# Autodesk Inventor assembly: Assemblyall
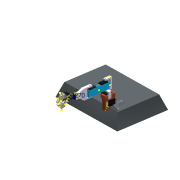
[picture p0: Inventor's stored thumbnail of the model, 180x180]
Saved by Autodesk Inventor 2022 (Build 260153000, 153)
## iProperties
Created: 2021-06-23
Part Number: Assemblyall
Document SubType Name: Assembly
Designer: athar
Author: athar
## Documents named in this file (16)
- C:\Users\Prajwal Patil\Desktop\HumanArmMimicBot-main\HumanArmMimicBot-main\AssemblyAlpha\Assemblyall.iam
- C:\Users\Prajwal Patil\Desktop\HumanArmMimicBot-main\HumanArmMimicBot-main\AssemblyAlpha\Part1_New.ipt
- C:\Users\Prajwal Patil\Desktop\HumanArmMimicBot-main\HumanArmMimicBot-main\AssemblyAlpha\Hand1.ipt
- C:\Users\Prajwal Patil\Desktop\HumanArmMimicBot-main\HumanArmMimicBot-main\AssemblyAlpha\Hand4.ipt
- C:\Users\Prajwal Patil\Desktop\HumanArmMimicBot-main\HumanArmMimicBot-main\AssemblyAlpha\Non Colour Claw.ipt
- C:\Users\Prajwal Patil\Desktop\HumanArmMimicBot-main\HumanArmMimicBot-main\AssemblyAlpha\Part1.ipt
- C:\Users\Prajwal Patil\Desktop\HumanArmMimicBot-main\HumanArmMimicBot-main\AssemblyAlpha\Part2.ipt
- C:\Users\Prajwal Patil\Desktop\HumanArmMimicBot-main\HumanArmMimicBot-main\AssemblyAlpha\Part4.ipt
- C:\Users\Prajwal Patil\Desktop\HumanArmMimicBot-main\HumanArmMimicBot-main\AssemblyAlpha\Part5.ipt
- C:\Users\Prajwal Patil\Desktop\HumanArmMimicBot-main\HumanArmMimicBot-main\AssemblyAlpha\motorshaft.ipt
- C:\Users\Prajwal Patil\Desktop\HumanArmMimicBot-main\HumanArmMimicBot-main\AssemblyAlpha\CSN EN ISO 8733 - 8x18-St.ipt
- C:\Users\Prajwal Patil\Desktop\HumanArmMimicBot-main\HumanArmMimicBot-main\AssemblyAlpha\Spur Gears2.iam
- C:\Users\Prajwal Patil\Desktop\HumanArmMimicBot-main\HumanArmMimicBot-main\AssemblyAlpha\bigServo_Derived.ipt
- C:\Users\Prajwal Patil\Desktop\HumanArmMimicBot-main\HumanArmMimicBot-main\AssemblyAlpha\Small_ServoDerived.ipt
- C:\Users\Prajwal Patil\Desktop\HumanArmMimicBot-main\HumanArmMimicBot-main\AssemblyAlpha\JIS B 1111 - M4x50.ipt
- C:\Users\Prajwal Patil\Desktop\HumanArmMimicBot-main\HumanArmMimicBot-main\AssemblyAlpha\base.ipt
## Components (68 placed, 15 different names)
1. Hand1:1 — Rotational:1, Rotational:2, Rotational:28, Mate:9, Rigid:18, Rotational:54
2. Hand4:1 — Rotational:2, Rotational:4, Rotational:9
3. Non Colour Claw:1 — Rotational:4, Rotational:5, Rotational:6
4. Part1:1 — Rigid:1, Rotational:26, Rotational:29, Rotational:30, Rotational:31, Rotational:59, Rotational:60, Rotational:61, Rotational:62
5. Part1_New:1 — Rotational:56, Rigid:3, Rotational:20, Rigid:7, Rotational:23, Rotational:24
6. Part2:1 — Rigid:1, Rotational:56, Rotational:25, Rotational:27, Rotational:40, Mate:10
7. Part4:1 — Rigid:3, Rigid:4, Rotational:18, Rotational:19, Mate:3, Mate:4, Rigid:9, Rigid:12
8. Part5:1 — Rigid:4, Rotational:16, Rotational:17, Rigid:19
9. Non Colour Claw:3 — Rotational:3, Rotational:7, Rotational:8
10. Hand4:2 — Rotational:1, Rotational:3, Rotational:10
11. motorshaft:1 — Rotational:16
12. motorshaft:3 — Rotational:23, Rotational:39
13. CSN EN ISO 8733 8x18-St:3 — Rotational:10
14. CSN EN ISO 8733 8x18-St:4 — Rotational:6
15. CSN EN ISO 8733 8x18-St:5 — Rotational:7, Rotational:55
16. CSN EN ISO 8733 8x18-St:6 — Rotational:9
17. CSN EN ISO 8733 8x18-St:7 — Rotational:8
18. CSN EN ISO 8733 8x18-St:8 — Rotational:5, Rotational:15
19. CSN EN ISO 8733 8x18-St:9 — Rotational:18
20. CSN EN ISO 8733 8x18-St:10 — Insert:1, Rotational:19
21. CSN EN ISO 8733 8x18-St:11 — Rigid:8
22. CSN EN ISO 8733 8x18-St:12 — Rotational:26
23. CSN EN ISO 8733 8x18-St:15 — Rigid:7
24. CSN EN ISO 8733 8x18-St:16 — Rotational:29
25. CSN EN ISO 8733 8x18-St:17 — Rotational:17, Rotational:48
26. CSN EN ISO 8733 8x18-St:18 — Insert:1
27. CSN EN ISO 8733 8x18-St:19 — Rotational:21
28. CSN EN ISO 8733 8x18-St:24 — Rotational:30, Rotational:57
29. CSN EN ISO 8733 8x18-St:25 — Rotational:28, Rotational:46
30. CSN EN ISO 8733 8x18-St:26 — Rotational:27
31. Spur Gears:1 [sub-assembly] — Rotational:52, Rotational:54
32. Spur Gears:2 [sub-assembly] — Rotational:51
33. Hand4:5 — Rotational:15, Rigid:8
34. motorshaft:5
35. motorshaft:6 — Rotational:20, Rotational:21
36. CSN EN ISO 8733 8x18-St:35 — Rotational:31, Rigid:20
37. CSN EN ISO 8733 8x18-St:36 — Rotational:25, Rotational:41
38. CSN EN ISO 8733 8x18-St:37 — Rotational:24
39. bigServo_Derived:1 — Mate:3, Mate:4, Rotational:32, Rigid:11
40. bigServo_Derived:3 — Rotational:36, Rotational:37, Rotational:39, Rigid:17, Mate:10
41. bigServo_Derived:4 — Rotational:41
42. Small_ServoDerived:1 — Rotational:46, Rigid:19, Rotational:47, Rotational:58, Rigid:21
43. Small_ServoDerived:2 — Mate:9, Rigid:15, Rigid:16, Rigid:18, Rotational:51
44. JIS B 1111 - M4x50:3 — Rigid:22
45. JIS B 1111 - M4x50:4 — Rigid:9
46. JIS B 1111 - M4x50:5 — Rigid:11
47. JIS B 1111 - M4x50:6 — Rotational:32
48. JIS B 1111 - M4x50:8 — Rigid:23
49. JIS B 1111 - M4x50:15 — Rigid:16
50. JIS B 1111 - M4x50:16 — Rigid:15, Rotational:42
51. JIS B 1111 - M4x50:17 — Rigid:12
52. JIS B 1111 - M4x50:18 — Rotational:36
53. JIS B 1111 - M4x50:21 — Rotational:37
54. base:1 — Rigid:20, Rotational:57
55. JIS B 1111 - M4x50:23 — Rigid:21
56. JIS B 1111 - M4x50:25 — Rigid:17
57. JIS B 1111 - M4x50:27 — Rotational:40
58. JIS B 1111 - M4x50:31 — Rotational:58
59. JIS B 1111 - M4x50:32 — Rotational:42
60. motorshaft:7 — Rotational:47
61. bigServo_Derived:5 — Rotational:48, Rotational:49, Rotational:50, Rigid:22, Rigid:23
62. JIS B 1111 - M4x50:33 — Rotational:50
63. JIS B 1111 - M4x50:35 — Rotational:49
64. Hand4:6 — Rotational:52, Rotational:55
65. JIS B 1111 - M4x50:36 — Rotational:59
66. JIS B 1111 - M4x50:37 — Rotational:61
67. JIS B 1111 - M4x50:38 — Rotational:62
68. JIS B 1111 - M4x50:39 — Rotational:60
## Relationships (71: RevoluteJoint 49, WeldJoint 17, Mate 4, Insert 1)
- Rigid:1 [WeldJoint] (-6.35 mm): Part1:1 ↔ Part2:1
- Rotational:56 [RevoluteJoint]: Part1_New:1 ↔ Part2:1
- Rigid:3 [WeldJoint]: Part1_New:1 ↔ Part4:1
- Rigid:4 [WeldJoint] (-4.7625 mm): Part4:1 ↔ Part5:1
- Rotational:1 [RevoluteJoint]: Hand1:1 ↔ Hand4:2
- Rotational:2 [RevoluteJoint]: Hand1:1 ↔ Hand4:1
- Rotational:3 [RevoluteJoint]: Non Colour Claw:3 ↔ Hand4:2
- Rotational:4 [RevoluteJoint]: Hand4:1 ↔ Non Colour Claw:1
- Insert:1: CSN EN ISO 8733 8x18-St:10 ↔ CSN EN ISO 8733 8x18-St:18
- Rotational:5 [RevoluteJoint]: Non Colour Claw:1 ↔ CSN EN ISO 8733 8x18-St:8
- Rotational:6 [RevoluteJoint]: Non Colour Claw:1 ↔ CSN EN ISO 8733 8x18-St:4
- Rotational:7 [RevoluteJoint]: Non Colour Claw:3 ↔ CSN EN ISO 8733 8x18-St:5
- Rotational:8 [RevoluteJoint]: Non Colour Claw:3 ↔ CSN EN ISO 8733 8x18-St:7
- Rotational:9 [RevoluteJoint] (-15.875 mm): Hand4:1 ↔ CSN EN ISO 8733 8x18-St:6
- Rotational:10 [RevoluteJoint] (1.5875 mm): Hand4:2 ↔ CSN EN ISO 8733 8x18-St:3
- Rotational:15 [RevoluteJoint] (-11.1125 mm): CSN EN ISO 8733 8x18-St:8 ↔ Hand4:5
- Rotational:16 [RevoluteJoint]: Part5:1 ↔ motorshaft:1
- Rotational:17 [RevoluteJoint] (-1.5875 mm): Part5:1 ↔ CSN EN ISO 8733 8x18-St:17
- Rotational:18 [RevoluteJoint]: Part4:1 ↔ CSN EN ISO 8733 8x18-St:9
- Rotational:19 [RevoluteJoint] (14.2875 mm): Part4:1 ↔ CSN EN ISO 8733 8x18-St:10
- Rotational:20 [RevoluteJoint] (44.45 mm): Part1_New:1 ↔ motorshaft:6
- Rotational:21 [RevoluteJoint] (-1.5875 mm): CSN EN ISO 8733 8x18-St:19 ↔ motorshaft:6
- Rigid:7 [WeldJoint] (3.175 mm): Part1_New:1 ↔ CSN EN ISO 8733 8x18-St:15
- Rotational:23 [RevoluteJoint]: Part1_New:1 ↔ motorshaft:3
- Rotational:24 [RevoluteJoint] (-3.175 mm): Part1_New:1 ↔ CSN EN ISO 8733 8x18-St:37
- Rotational:25 [RevoluteJoint] (3.175 mm): Part2:1 ↔ CSN EN ISO 8733 8x18-St:36
- Rotational:26 [RevoluteJoint] (-1.5875 mm): Part1:1 ↔ CSN EN ISO 8733 8x18-St:12
- Rotational:27 [RevoluteJoint] (4.7625 mm): Part2:1 ↔ CSN EN ISO 8733 8x18-St:26
- Rotational:28 [RevoluteJoint] (15.875 mm): Hand1:1 ↔ CSN EN ISO 8733 8x18-St:25
- Rotational:29 [RevoluteJoint] (-3.175 mm): Part1:1 ↔ CSN EN ISO 8733 8x18-St:16
- Rotational:30 [RevoluteJoint] (14.2875 mm): Part1:1 ↔ CSN EN ISO 8733 8x18-St:24
- Rotational:31 [RevoluteJoint] (12.7 mm): Part1:1 ↔ CSN EN ISO 8733 8x18-St:35
- Rigid:8 [WeldJoint] (-11.1125 mm): CSN EN ISO 8733 8x18-St:11 ↔ Hand4:5
- Mate:3: Part4:1 ↔ bigServo_Derived:1
- Mate:4: Part4:1 ↔ bigServo_Derived:1
- Mate:9: Hand1:1 ↔ Small_ServoDerived:2
- Rigid:9 [WeldJoint] (9.525 mm): Part4:1 ↔ JIS B 1111 - M4x50:4
- Rotational:32 [RevoluteJoint] (11.1125 mm): bigServo_Derived:1 ↔ JIS B 1111 - M4x50:6
- Rigid:11 [WeldJoint] (11.1125 mm): bigServo_Derived:1 ↔ JIS B 1111 - M4x50:5
- Rigid:12 [WeldJoint] (9.525 mm): Part4:1 ↔ JIS B 1111 - M4x50:17
- Rigid:15 [WeldJoint] (-14.2875 mm): Small_ServoDerived:2 ↔ JIS B 1111 - M4x50:16
- Rigid:16 [WeldJoint] (9.525 mm): Small_ServoDerived:2 ↔ JIS B 1111 - M4x50:15
- Rotational:36 [RevoluteJoint] (11.1125 mm): bigServo_Derived:3 ↔ JIS B 1111 - M4x50:18
- Rotational:37 [RevoluteJoint] (12.7 mm): bigServo_Derived:3 ↔ JIS B 1111 - M4x50:21
- Rotational:39 [RevoluteJoint] (-41.275 mm): motorshaft:3 ↔ bigServo_Derived:3
- Rigid:17 [WeldJoint] (12.7 mm): bigServo_Derived:3 ↔ JIS B 1111 - M4x50:25
- Rotational:40 [RevoluteJoint] (6.35 mm): Part2:1 ↔ JIS B 1111 - M4x50:27
- Rotational:41 [RevoluteJoint]: CSN EN ISO 8733 8x18-St:36 ↔ bigServo_Derived:4
- Rotational:42 [RevoluteJoint] (12.7 mm): JIS B 1111 - M4x50:16 ↔ JIS B 1111 - M4x50:32
- Rigid:18 [WeldJoint] (9.525 mm): Hand1:1 ↔ Small_ServoDerived:2
- Rotational:46 [RevoluteJoint]: CSN EN ISO 8733 8x18-St:25 ↔ Small_ServoDerived:1
- Rigid:19 [WeldJoint] (-4.7625 mm): Part5:1 ↔ Small_ServoDerived:1
- Rotational:47 [RevoluteJoint] (42.8625 mm): Small_ServoDerived:1 ↔ motorshaft:7
- Rotational:48 [RevoluteJoint] (9.525 mm): CSN EN ISO 8733 8x18-St:17 ↔ bigServo_Derived:5
- Rotational:49 [RevoluteJoint] (11.1125 mm): bigServo_Derived:5 ↔ JIS B 1111 - M4x50:35
- Rotational:50 [RevoluteJoint] (11.1125 mm): bigServo_Derived:5 ↔ JIS B 1111 - M4x50:33
- Rotational:51 [RevoluteJoint] (-7.9375 mm): Spur Gears:2 ↔ Small_ServoDerived:2
- Rotational:52 [RevoluteJoint] (-7.9375 mm): Spur Gears:1 ↔ Hand4:6
- Rotational:54 [RevoluteJoint] (-15.875 mm): Hand1:1 ↔ Spur Gears:1
- Rotational:55 [RevoluteJoint] (3.175 mm): CSN EN ISO 8733 8x18-St:5 ↔ Hand4:6
- Rigid:20 [WeldJoint]: CSN EN ISO 8733 8x18-St:35 ↔ base:1
- Rotational:57 [RevoluteJoint]: CSN EN ISO 8733 8x18-St:24 ↔ base:1
- Rotational:58 [RevoluteJoint] (11.1125 mm): Small_ServoDerived:1 ↔ JIS B 1111 - M4x50:31
- Rigid:21 [WeldJoint] (7.9375 mm): Small_ServoDerived:1 ↔ JIS B 1111 - M4x50:23
- Mate:10: Part2:1 ↔ bigServo_Derived:3
- Rigid:22 [WeldJoint] (-11.1125 mm): JIS B 1111 - M4x50:3 ↔ bigServo_Derived:5
- Rigid:23 [WeldJoint] (10.16 mm): JIS B 1111 - M4x50:8 ↔ bigServo_Derived:5
- Rotational:59 [RevoluteJoint] (11.1125 mm): Part1:1 ↔ JIS B 1111 - M4x50:36
- Rotational:60 [RevoluteJoint] (11.1125 mm): Part1:1 ↔ JIS B 1111 - M4x50:39
- Rotational:61 [RevoluteJoint] (11.1125 mm): Part1:1 ↔ JIS B 1111 - M4x50:37
- Rotational:62 [RevoluteJoint] (11.1125 mm): Part1:1 ↔ JIS B 1111 - M4x50:38
